# Autodesk Inventor assembly: Meca500 Assembly simple
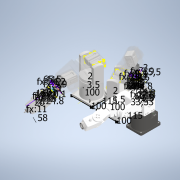
[picture p0: Inventor's stored thumbnail of the model, 180x180]
Saved by Autodesk Inventor 2020.2 (Build 242310000, 310)
## iProperties
Created: 2018-03-09
Part Number: Meca500 Assembly simple
Document SubType Name: Assembly
Designer: JochenAlt
Sending System: Autodesk Inventor 2018
Preprocessor: ST-DEVELOPER v16.13
Title: C:\SVN\Mechanical\Meca500\Meca500 Step files\Meca500 - Assembly simple.stp
Author: Jonathan
## Documents named in this file (9)
- D:\Projects\Gerhard\CAD\extern\Meca500\Meca500 Assembly simple.iam
- D:\Projects\Gerhard\CAD\extern\Meca500\Axis 1 - Base assembly simple.ipt
- D:\Projects\Gerhard\CAD\extern\Meca500\Axis 2 - Hip support simple.ipt
- D:\Projects\Gerhard\CAD\extern\Meca500\Axis 3 - Lower arm simple.ipt
- D:\Projects\Gerhard\CAD\extern\Meca500\A⁮xis 4 - Elbow simple.ipt
- D:\Projects\Gerhard\CAD\extern\Meca500\Axis 5 - Wrist support simple.ipt
- D:\Projects\Gerhard\CAD\extern\Meca500\Axis 6 - Wrist simple v3.ipt
- D:\Projects\Gerhard\CAD\Arm.iam
- D:\Projects\Gerhard\CAD\Arm HD.iam
## Components (8 placed, 7 different names)
1. Axis 1 - Base assembly simple:1 — Passend:9, Passend:10, Fluchtend:1, Fluchtend:2, Passend:12
2. Axis 2 - Hip support simple:1 — Passend:8, Passend:9, Passend:10, Passend:11
3. Axis 3 - Lower arm simple:1 — Passend:6, Passend:7, Passend:8, Passend:11
4. A⁮xis 4 - Elbow simple:1 — Passend:4, Passend:5, Passend:6, Passend:7
5. Axis 5 - Wrist support simple:1 — Passend:2, Passend:3, Passend:4, Passend:5
6. Axis 6 - Wrist simple v3:1 — Passend:2, Passend:3
7. Arm:1 [sub-assembly] — Fluchtend:1, Fluchtend:2, Passend:12, Fluchtend:3, Fluchtend:4, Passend:13
8. Arm:2 [sub-assembly] — Fluchtend:3, Fluchtend:4, Passend:13
## Relationships (16: Mate 12, Flush 4)
- Passend:2 [Mate]: Axis 5 - Wrist support simple:1 ↔ Axis 6 - Wrist simple v3:1
- Passend:3 [Mate]: Axis 5 - Wrist support simple:1 ↔ Axis 6 - Wrist simple v3:1
- Passend:4 [Mate]: A⁮xis 4 - Elbow simple:1 ↔ Axis 5 - Wrist support simple:1
- Passend:5 [Mate]: A⁮xis 4 - Elbow simple:1 ↔ Axis 5 - Wrist support simple:1
- Passend:6 [Mate]: Axis 3 - Lower arm simple:1 ↔ A⁮xis 4 - Elbow simple:1
- Passend:7 [Mate]: Axis 3 - Lower arm simple:1 ↔ A⁮xis 4 - Elbow simple:1
- Passend:8 [Mate]: Axis 2 - Hip support simple:1 ↔ Axis 3 - Lower arm simple:1
- Passend:9 [Mate]: Axis 1 - Base assembly simple:1 ↔ Axis 2 - Hip support simple:1
- Passend:10 [Mate]: Axis 1 - Base assembly simple:1 ↔ Axis 2 - Hip support simple:1
- Passend:11 [Mate]: Axis 2 - Hip support simple:1 ↔ Axis 3 - Lower arm simple:1
- Fluchtend:1 [Flush]: Axis 1 - Base assembly simple:1 ↔ Arm:1
- Fluchtend:2 [Flush]: Axis 1 - Base assembly simple:1 ↔ Arm:1
- Passend:12 [Mate] (50 mm): Axis 1 - Base assembly simple:1 ↔ Arm:1
- Fluchtend:3 [Flush]: Arm:1 ↔ Arm:2
- Fluchtend:4 [Flush]: Arm:1 ↔ Arm:2
- Passend:13 [Mate] (30 mm): Arm:1 ↔ Arm:2
